# Autodesk Inventor assembly: Omni Full 4in_MIR
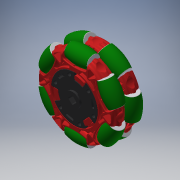
[picture p0: Inventor's stored thumbnail of the model, 180x180]
Saved by Autodesk Inventor 2016 (Build 200138000, 138)
## iProperties
Created: 2019-01-03
Part Number: Omni Full 4in_MIR
Document SubType Name: Assembly
Designer: Afnan
Author: Afnan
## Documents named in this file (4)
- D:\New Laptop\(1) New Laptop\AFNAN ALI flashdrive backup\VEXPARTS\Vex parts\VEXPRO\Wheels\Omni\Omni Full 4in_MIR.iam
- D:\New Laptop\(1) New Laptop\AFNAN ALI flashdrive backup\VEXPARTS\Vex parts\VEXPRO\Wheels\Omni\4_Omni-Directional_Wheel_v2_276-6194_MIR.ipt
- D:\New Laptop\(1) New Laptop\AFNAN ALI flashdrive backup\VEXPARTS\Vex parts\VEXPRO\Wheels\Wheel Hub_MIR.ipt
- D:\New Laptop\(1) New Laptop\AFNAN ALI flashdrive backup\VEXPARTS\Vex parts\VEXPRO\Wheels\Hex to Square 0.25in_MIR.ipt
## Components (5 placed, 3 different names)
1. 4_Omni-Directional_Wheel_v2_276-6194_MIR:1 — Mate:3, Mate:2, Mate:1, Mate:6, Mate:5, Mate:4
2. Wheel Hub_MIR:1 — Mate:3, Mate:2, Mate:1, Mate:10
3. Wheel Hub_MIR:2 — Mate:6, Mate:5, Mate:4, Mate:9, Mate:8, Mate:7
4. Hex to Square 0.25in_MIR:1 — Mate:9, Mate:8, Mate:7, Mate:12, Mate:11
5. Hex to Square 0.25in_MIR:2 — Mate:12, Mate:11, Mate:10
## Relationships (12: Mate 12)
- Mate:3: 4_Omni-Directional_Wheel_v2_276-6194_MIR:1 ↔ Wheel Hub_MIR:1
- Mate:2: 4_Omni-Directional_Wheel_v2_276-6194_MIR:1 ↔ Wheel Hub_MIR:1
- Mate:1: 4_Omni-Directional_Wheel_v2_276-6194_MIR:1 ↔ Wheel Hub_MIR:1
- Mate:6: 4_Omni-Directional_Wheel_v2_276-6194_MIR:1 ↔ Wheel Hub_MIR:2
- Mate:5: 4_Omni-Directional_Wheel_v2_276-6194_MIR:1 ↔ Wheel Hub_MIR:2
- Mate:4: 4_Omni-Directional_Wheel_v2_276-6194_MIR:1 ↔ Wheel Hub_MIR:2
- Mate:9: Wheel Hub_MIR:2 ↔ Hex to Square 0.25in_MIR:1
- Mate:8: Wheel Hub_MIR:2 ↔ Hex to Square 0.25in_MIR:1
- Mate:7: Wheel Hub_MIR:2 ↔ Hex to Square 0.25in_MIR:1
- Mate:12: Hex to Square 0.25in_MIR:1 ↔ Hex to Square 0.25in_MIR:2
- Mate:11: Hex to Square 0.25in_MIR:1 ↔ Hex to Square 0.25in_MIR:2
- Mate:10: Wheel Hub_MIR:1 ↔ Hex to Square 0.25in_MIR:2
